# Autodesk Inventor assembly: Structure
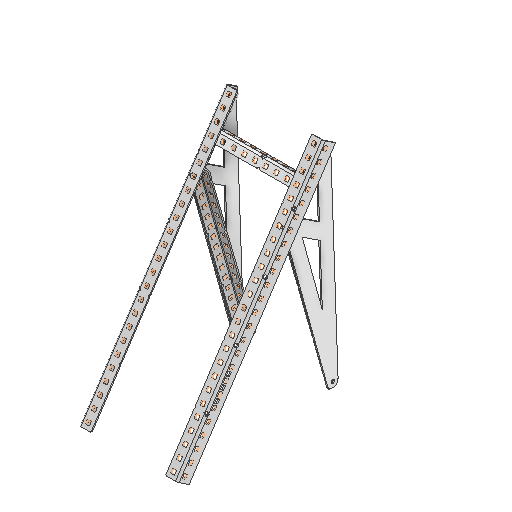
[picture p0: Inventor's stored thumbnail of the model, 512x512]
Saved by Autodesk Inventor 2025 (Build 290162000, 162)
## iProperties
Created: 2025-02-15
Part Number: Structure
Document SubType Name: Assembly
Designer: Averey Ku
Author: Averey Ku
## Documents named in this file (6)
- D:\VEX\High Stakes\CAD\V5\Conveyer\Structure.iam
- D:\VEX\High Stakes\CAD\ROBOPROS-CAD-Inventor\Structure\C Channel\Aluminum 1x3x1 Half Thick Cut\Alu C Half Thick 1x3x1x25.ipt
- D:\VEX\High Stakes\CAD\ROBOPROS-CAD-Inventor\Structure\Angle\Aluminum 1x1\Alu Angle 1x1x16.ipt
- D:\VEX\High Stakes\CAD\V5\Conveyer\Custom Parts\Triangle Gusset.ipt
- D:\VEX\High Stakes\CAD\ROBOPROS-CAD-Inventor\Motion\Shaft LS\Bearing Flat Low Profile.ipt
- D:\VEX\High Stakes\CAD\ROBOPROS-CAD-Inventor\Structure\Angle\Aluminum 1x1\Alu Angle 1x1x9.ipt
## Components (9 placed, 5 different names)
1. Alu C Half Thick 1x3x1x25:1 — Mate:9
2. Alu C Half Thick 1x3x1x25:2 — Insert:6
3. Alu Angle 1x1x16:1 — Mate:7
4. Alu Angle 1x1x16:2 — Mate:8
5. Triangle Gusset:1 — Mate:7
6. Triangle Gusset:2 — Mate:8
7. Bearing Flat Low Profile:1
8. Bearing Flat Low Profile:2
9. Alu Angle 1x1x9:1 — Insert:6, Mate:9
## Relationships (15: Mate 9, Insert 6)
- [Mate]: Alu C Half Thick 1x3x1x25:1 ↔ Alu C Half Thick 1x3x1x25:2
- [Insert] (1.5875 mm): Alu C Half Thick 1x3x1x25:2 ↔ Alu Angle 1x1x16:1
- [Insert] (1.5875 mm): Alu C Half Thick 1x3x1x25:1 ↔ Alu Angle 1x1x16:2
- [Mate]: Alu Angle 1x1x16:1 ↔ Triangle Gusset:1
- [Mate]: Alu C Half Thick 1x3x1x25:2 ↔ Triangle Gusset:1
- [Insert]: Alu C Half Thick 1x3x1x25:1 ↔ Triangle Gusset:2
- [Mate]: Alu C Half Thick 1x3x1x25:1 ↔ Triangle Gusset:2
- [Insert] (1.5875 mm): Alu C Half Thick 1x3x1x25:2 ↔ Bearing Flat Low Profile:1
- [Mate]: Alu C Half Thick 1x3x1x25:2 ↔ Bearing Flat Low Profile:1
- [Insert] (1.5875 mm): Alu C Half Thick 1x3x1x25:1 ↔ Bearing Flat Low Profile:2
- [Mate]: Alu C Half Thick 1x3x1x25:1 ↔ Bearing Flat Low Profile:2
- Mate:7: Alu Angle 1x1x16:1 ↔ Triangle Gusset:1
- Mate:8: Alu Angle 1x1x16:2 ↔ Triangle Gusset:2
- Insert:6: Alu C Half Thick 1x3x1x25:2 ↔ Alu Angle 1x1x9:1
- Mate:9: Alu C Half Thick 1x3x1x25:1 ↔ Alu Angle 1x1x9:1
